# Autodesk Inventor assembly: Assembly_XYTable_Aliepexress
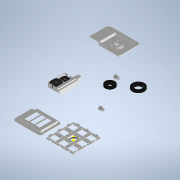
[picture p0: Inventor's stored thumbnail of the model, 180x180]
Saved by Autodesk Inventor 2022 (Build 260153000, 153)
## iProperties
Created: 2021-11-18
Part Number: Assembly_XYTable_Aliepexress
Document SubType Name: Assembly
Designer: diederichbenedict
Author: diederichbenedict
## Documents named in this file (11)
- C:\Users\diederichbenedict\Dropbox\Dokumente\Promotion\PROJECTS\UC2\02_CAD\INVENTOR\uc2_v3\Assembly_XYTable_Aliepexress.iam
- C:\Users\diederichbenedict\Dropbox\Dokumente\Promotion\PROJECTS\UC2\02_CAD\INVENTOR\uc2_v3\10_Base_puzzle_v3.ipt
- C:\Users\diederichbenedict\Dropbox\Dokumente\Promotion\PROJECTS\UC2\02_CAD\INVENTOR\uc2_v3\30_XYTabel_Aliexpress_basplateadapter.ipt
- C:\Users\diederichbenedict\Dropbox\Dokumente\Promotion\PROJECTS\UC2\02_CAD\INVENTOR\uc2_v3\30_XYTable_Aliexpress_sampleinsert.ipt
- C:\Users\diederichbenedict\Dropbox\Dokumente\Promotion\PROJECTS\UC2\02_CAD\INVENTOR\uc2_v3\30_XYTable_Aliexpress_motormount.ipt
- C:\Users\diederichbenedict\Dropbox\Dokumente\Promotion\PROJECTS\UC2\02_CAD\INVENTOR\uc2_v3\00_NEMA17_pancake.iam
- C:\Users\diederichbenedict\Dropbox\Dokumente\Promotion\PROJECTS\UC2\02_CAD\INVENTOR\uc2_v3\00_XYTable_medium_gear.ipt
- C:\Users\diederichbenedict\Dropbox\Dokumente\Promotion\PROJECTS\UC2\02_CAD\INVENTOR\uc2_v3\00_XYTable_pulley.ipt
- C:\Users\diederichbenedict\Dropbox\Dokumente\Promotion\PROJECTS\UC2\02_CAD\INVENTOR\uc2_v3\00_XYTable_large_gear.ipt
- C:\Users\diederichbenedict\Dropbox\Dokumente\Promotion\PROJECTS\UC2\02_CAD\INVENTOR\uc2_v3\30_XYTable_Aliexpress_sampleinsert_round.ipt
- C:\Users\diederichbenedict\Dropbox\Dokumente\Promotion\PROJECTS\UC2\02_CAD\INVENTOR\uc2_v3\SMLM_Holder\SMLM_Holder_v1.iam
## Components (12 placed, 10 different names)
1. 10_Base_puzzle_v3:1 — Flush:1
2. 30_XYTabel_Aliexpress_basplateadapter:1 — Flush:1, Mate:4
3. 30_XYTable_Aliexpress_sampleinsert:1 — Mate:4
4. 30_XYTable_Aliexpress_motormount:1 — Einfügen:1, Winkel:1, Einfügen:2, Winkel:2
5. 00_NEMA17_pancake:1 [sub-assembly] — Einfügen:1, Winkel:1
6. 00_NEMA17_pancake:2 [sub-assembly] — Einfügen:2, Winkel:2
7. 00_XYTable_medium_gear:1
8. 00_XYTable_pulley:1
9. 00_XYTable_large_gear:1
10. 00_XYTable_pulley:2
11. 30_XYTable_Aliexpress_sampleinsert_round:1 — Einfügen:3
12. SMLM_Holder_v1:1 [sub-assembly] — Einfügen:3
## Relationships (7: Insert 3, Angle 2, Flush 1, Mate 1)
- Flush:1: 10_Base_puzzle_v3:1 ↔ 30_XYTabel_Aliexpress_basplateadapter:1
- Mate:4 (-11.185 mm): 30_XYTabel_Aliexpress_basplateadapter:1 ↔ 30_XYTable_Aliexpress_sampleinsert:1
- Einfügen:1 [Insert]: 30_XYTable_Aliexpress_motormount:1 ↔ 00_NEMA17_pancake:1
- Winkel:1 [Angle] (0 deg): 30_XYTable_Aliexpress_motormount:1 ↔ 00_NEMA17_pancake:1
- Einfügen:2 [Insert]: 30_XYTable_Aliexpress_motormount:1 ↔ 00_NEMA17_pancake:2
- Winkel:2 [Angle] (0 deg): 30_XYTable_Aliexpress_motormount:1 ↔ 00_NEMA17_pancake:2
- Einfügen:3 [Insert]: 30_XYTable_Aliexpress_sampleinsert_round:1 ↔ SMLM_Holder_v1:1
